# Autodesk Inventor assembly: 0904_right_leg
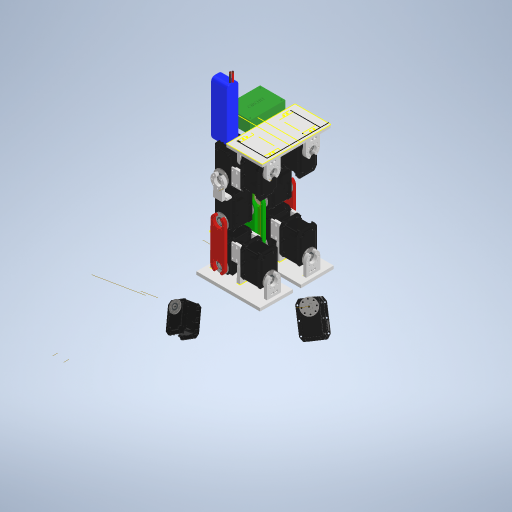
[picture p0: Inventor's stored thumbnail of the model, 512x512]
Saved by Autodesk Inventor 2024.3 (Build 283343000, 343)
## iProperties
Created: 2024-09-03
Part Number: 0904_right_leg
Document SubType Name: Assembly
Designer: gretc
Author: gretc
## Documents named in this file (33)
- C:\Users\gretc\Desktop\inventor_part\0904_right_leg.iam
- C:\Users\gretc\Desktop\inventor_part\다이나믹셀\MX-106T+idle.ipt.iam
- C:\Users\gretc\Desktop\inventor_part\다이나믹셀\MX-64T+idle.ipt.iam
- C:\Users\gretc\Desktop\inventor_part\혼\64-106Horn.ipt
- C:\Users\gretc\Desktop\inventor_part\0904_joint.ipt
- C:\Users\gretc\Desktop\inventor_part\0904_thigh_1.ipt
- C:\Users\gretc\Desktop\inventor_part\0904_thigh_2.ipt
- C:\Users\gretc\Desktop\inventor_part\0904_106-64_adt.ipt
- C:\Users\gretc\Desktop\inventor_part\0904_foot_adt.ipt
- C:\Users\gretc\Desktop\inventor_part\0904_foot-106-adt.ipt
- C:\Users\gretc\Desktop\inventor_part\0904-foot.ipt
- C:\Users\gretc\Desktop\inventor_part\아이들러\64아이들러.iam
- C:\Users\gretc\Desktop\inventor_part\0904-idler-supporter.ipt
- C:\Users\gretc\Desktop\inventor_part\0904_right_foot.ipt
- C:\Users\gretc\Desktop\inventor_part\다이나믹셀\MX-106T+idle.ipt_MIR.iam
- C:\Users\gretc\Desktop\inventor_part\다이나믹셀\MX-64T+idle.ipt_MIR.iam
- C:\Users\gretc\Desktop\inventor_part\혼\64-106Horn_MIR.ipt
- C:\Users\gretc\Desktop\inventor_part\0904_joint_MIR.ipt
- C:\Users\gretc\Desktop\inventor_part\0904_thigh_1_MIR.ipt
- C:\Users\gretc\Desktop\inventor_part\0904_thigh_2_MIR.ipt
- C:\Users\gretc\Desktop\inventor_part\0904_106-64_adt_MIR1.ipt
- C:\Users\gretc\Desktop\inventor_part\0904_foot_adt_MIR.ipt
- C:\Users\gretc\Desktop\inventor_part\아이들러\64아이들러_MIR.iam
- C:\Users\gretc\Desktop\inventor_part\0904-idler-supporter_MIR1.ipt
- C:\Users\gretc\Desktop\inventor_part\0904_right_foot_MIR.ipt
- C:\Users\gretc\Desktop\inventor_part\Power_Control_inventor\Circuit.ipt
- C:\Users\gretc\Desktop\inventor_part\Power_Control_inventor\Enrichpower_2200mAh_11.1V_30C.ipt
- C:\Users\gretc\Desktop\inventor_part\0904_robot_bodyframe1.ipt
- C:\Users\gretc\Desktop\inventor_part\다이나믹셀\MX-28T_R+idle.ipt.iam
- C:\Users\gretc\Desktop\inventor_part\혼\28Horn.ipt
- MX-106T+idle.ipt
- MX-64T+idle.ipt
- MX-28T_R+idle.ipt
## Components (60 placed, 29 different names)
1. MX-106T+idle.ipt:1 [sub-assembly] — 회전:1, 플러쉬:1, 플러쉬:3, 메이트:1, 플러쉬:5, 플러쉬:6, 플러쉬:12, 플러쉬:13, 플러쉬:14, 플러쉬:15, 플러쉬:16
2. MX-64T+idle.ipt:1 [sub-assembly] — 회전:2, 플러쉬:9, 플러쉬:10, 메이트:4, 메이트:15, 삽입:4
3. 64-106Horn:1 — 회전:1, 플러쉬:11, 회전:6
4. 64-106Horn:2 — 회전:2, 삽입:3, 메이트:18, 메이트:21
5. MX-106T+idle.ipt:2 [sub-assembly] — 플러쉬:1, 플러쉬:2, 플러쉬:3, 플러쉬:4, 플러쉬:6, 메이트:2, 플러쉬:9, 플러쉬:10, 메이트:4, 회전:9, 메이트:22, 삽입:5, 메이트:118
6. 64-106Horn:3 — 플러쉬:17
7. MX-106T+idle.ipt:3 [sub-assembly] — 플러쉬:2, 플러쉬:4, 플러쉬:5, 플러쉬:7, 메이트:3, 플러쉬:8, 플러쉬:18, 플러쉬:19, 회전:8, 플러쉬:21, 플러쉬:25, 플러쉬:26, 메이트:25, 메이트:26, 메이트:35
8. 64-106Horn:4 — 메이트:5, 메이트:6, 회전:7
9. 64-106Horn:5 — 회전:5, 메이트:9, 메이트:10, 삽입:1
10. MX-64T+idle.ipt:2 [sub-assembly] — 플러쉬:7, 메이트:3, 플러쉬:8, 회전:5, 플러쉬:20
11. 0904_joint:1 — 플러쉬:11, 플러쉬:12
12. 0904_joint:2 — 회전:6, 회전:7, 각도:2, 플러쉬:29
13. 0904_thigh_1:1 — 플러쉬:13, 플러쉬:14
14. 0904_thigh_2:1 — 플러쉬:15, 플러쉬:16, 플러쉬:17
15. 0904_106-64_adt:1 — 플러쉬:18, 플러쉬:19
16. 0904_foot_adt:1 — 플러쉬:20, 플러쉬:23, 플러쉬:24
17. 0904_106-64_adt:2 — 회전:8
18. 0904_106-64_adt:3 — 회전:9
19. 0904_foot_adt:2 — 삽입:1, 플러쉬:27, 플러쉬:28
20. 0904_foot-106-adt:1 — 플러쉬:21
21. 0904_foot_adt:4 — 삽입:3, 메이트:19, 플러쉬:22
22. 0904_foot_adt:5 — 삽입:4, 메이트:16, 플러쉬:22
23. 0904_106-64_adt:4 — 메이트:23, 삽입:5
24. 0904-foot:1 — 플러쉬:23, 플러쉬:24
25. 64아이들러:1 [sub-assembly] — 메이트:28, 메이트:29, 메이트:30, 메이트:31, 메이트:32, 메이트:38, 삽입:6, 메이트:43, 메이트:45
26. 0904-idler-supporter:1 — 플러쉬:25, 플러쉬:26, 메이트:27, 메이트:29
27. 0904_foot_adt:6 — 메이트:40, 삽입:6, 각도:2, 메이트:48
28. 0904_right_foot:1 — 플러쉬:27, 플러쉬:28
29. MX-106T+idle.ipt_MIR:1 [sub-assembly] — 메이트:72, 플러쉬:33, 플러쉬:34, 플러쉬:35, 플러쉬:36, 메이트:77, 메이트:79, 메이트:80, 메이트:82, 메이트:83, 회전:10
30. MX-64T+idle.ipt_MIR:1 [sub-assembly] — 메이트:73, 플러쉬:30, 플러쉬:31, 메이트:87, 삽입:8, 회전:11
31. 64-106Horn_MIR:1 — 메이트:78, 회전:10, 회전:15
32. 64-106Horn_MIR:2 — 삽입:7, 메이트:90, 메이트:93, 회전:11
33. MX-106T+idle.ipt_MIR:2 [sub-assembly] — 메이트:73, 플러쉬:30, 플러쉬:31, 플러쉬:32, 플러쉬:33, 플러쉬:34, 플러쉬:35, 플러쉬:37, 플러쉬:38, 삽입:9, 메이트:94, 회전:12, 회전:17, 메이트:119
34. 64-106Horn_MIR:3 — 메이트:81, 회전:12
35. MX-106T+idle.ipt_MIR:3 [sub-assembly] — 플러쉬:36, 플러쉬:37, 플러쉬:38, 플러쉬:39, 메이트:74, 플러쉬:40, 메이트:84, 메이트:85, 메이트:98, 메이트:99, 메이트:100, 메이트:101, 메이트:107, 회전:13, 회전:16
36. 64-106Horn_MIR:4 — 메이트:75, 메이트:76, 회전:13, 회전:14
37. MX-64T+idle.ipt_MIR:2 [sub-assembly] — 플러쉬:39, 메이트:74, 플러쉬:40, 메이트:86
38. 0904_joint_MIR:1 — 메이트:77, 메이트:78
39. 0904_joint_MIR:2 — 각도:3, 메이트:117, 회전:14, 회전:15
40. 0904_thigh_1_MIR:1 — 메이트:79, 메이트:80
41. 0904_thigh_2_MIR:1 — 메이트:81, 메이트:82, 메이트:83
42. 0904_106-64_adt_MIR1:1 — 메이트:84, 메이트:85
43. 0904_foot_adt_MIR:1 — 메이트:86
44. 0904_106-64_adt_MIR1:2 — 회전:16
45. 0904_106-64_adt_MIR1:3 — 회전:17
46. 0904_foot_adt_MIR:2 — 메이트:115, 메이트:116
47. 0904_foot_adt_MIR:3 — 삽입:7, 플러쉬:41, 메이트:92, 플러쉬:42, 플러쉬:43
48. 0904_foot_adt_MIR:4 — 플러쉬:41, 삽입:8, 메이트:89
49. 0904_106-64_adt_MIR1:4 — 삽입:9, 메이트:96
50. 64아이들러_MIR:1 [sub-assembly] — 메이트:97, 메이트:103, 메이트:104, 메이트:105, 메이트:106, 삽입:10, 메이트:108, 메이트:111, 메이트:113
51. 0904-idler-supporter_MIR1:1 — 메이트:97, 메이트:98, 메이트:99, 메이트:102
52. 0904_foot_adt_MIR:5 — 각도:3, 삽입:10, 메이트:109, 메이트:114
53. 0904_right_foot_MIR:1 — 메이트:115, 메이트:116
54. Circuit:1 — 메이트:118
55. Enrichpower_2200mAh_11.1V_30C:1 — 메이트:119
56. 0904_robot_bodyframe1:1 — 플러쉬:42, 플러쉬:43
57. MX-28T_R+idle.ipt:1 [sub-assembly] — 메이트:120, 메이트:123
58. MX-64T+idle.ipt:3 [sub-assembly] — 메이트:129, 메이트:132
59. 28Horn:1 — 메이트:121, 메이트:123, 메이트:124
60. 64-106Horn:6 — 메이트:130, 메이트:132
## Relationships (165: Mate 92, Flush 43, RevoluteJoint 17, Insert 9, Angle 4)
- 회전:1 [RevoluteJoint]: MX-106T+idle.ipt:1 ↔ 64-106Horn:1
- 회전:2 [RevoluteJoint]: MX-64T+idle.ipt:1 ↔ 64-106Horn:2
- [RevoluteJoint]: MX-106T+idle.ipt:2 ↔ 64-106Horn:3
- [RevoluteJoint]: MX-106T+idle.ipt:3 ↔ 64-106Horn:4
- 플러쉬:1 [Flush]: MX-106T+idle.ipt:1 ↔ MX-106T+idle.ipt:2
- 플러쉬:2 [Flush]: MX-106T+idle.ipt:2 ↔ MX-106T+idle.ipt:3
- 플러쉬:3 [Flush]: MX-106T+idle.ipt:1 ↔ MX-106T+idle.ipt:2
- 플러쉬:4 [Flush]: MX-106T+idle.ipt:2 ↔ MX-106T+idle.ipt:3
- 메이트:1 [Mate]: MX-106T+idle.ipt:1
- 플러쉬:5 [Flush] (75 mm): MX-106T+idle.ipt:1 ↔ MX-106T+idle.ipt:3
- 플러쉬:6 [Flush] (75 mm): MX-106T+idle.ipt:1 ↔ MX-106T+idle.ipt:2
- 메이트:2 [Mate]: MX-106T+idle.ipt:2
- 플러쉬:7 [Flush]: MX-106T+idle.ipt:3 ↔ MX-64T+idle.ipt:2
- 메이트:3 [Mate]: MX-106T+idle.ipt:3 ↔ MX-64T+idle.ipt:2
- 플러쉬:8 [Flush] (50 mm): MX-106T+idle.ipt:3 ↔ MX-64T+idle.ipt:2
- 회전:5 [RevoluteJoint]: 64-106Horn:5 ↔ MX-64T+idle.ipt:2
- 플러쉬:9 [Flush]: MX-64T+idle.ipt:1 ↔ MX-106T+idle.ipt:2
- 플러쉬:10 [Flush] (50 mm): MX-64T+idle.ipt:1 ↔ MX-106T+idle.ipt:2
- 메이트:4 [Mate] (-35 mm): MX-64T+idle.ipt:1 ↔ MX-106T+idle.ipt:2
- 메이트:5 [Mate]: 64-106Horn:4
- 메이트:6 [Mate]: 64-106Horn:4
- 플러쉬:11 [Flush]: 64-106Horn:1 ↔ 0904_joint:1
- 플러쉬:12 [Flush]: MX-106T+idle.ipt:1 ↔ 0904_joint:1
- 회전:6 [RevoluteJoint]: 64-106Horn:1 ↔ 0904_joint:2
- 회전:7 [RevoluteJoint]: 64-106Horn:4 ↔ 0904_joint:2
- 플러쉬:13 [Flush]: MX-106T+idle.ipt:1 ↔ 0904_thigh_1:1
- 플러쉬:14 [Flush]: MX-106T+idle.ipt:1 ↔ 0904_thigh_1:1
- 플러쉬:15 [Flush]: MX-106T+idle.ipt:1 ↔ 0904_thigh_2:1
- 플러쉬:16 [Flush]: MX-106T+idle.ipt:1 ↔ 0904_thigh_2:1
- 플러쉬:17 [Flush]: 64-106Horn:3 ↔ 0904_thigh_2:1
- 플러쉬:18 [Flush]: MX-106T+idle.ipt:3 ↔ 0904_106-64_adt:1
- 플러쉬:19 [Flush]: MX-106T+idle.ipt:3 ↔ 0904_106-64_adt:1
- 플러쉬:20 [Flush]: MX-64T+idle.ipt:2 ↔ 0904_foot_adt:1
- 회전:8 [RevoluteJoint]: MX-106T+idle.ipt:3 ↔ 0904_106-64_adt:2
- 회전:9 [RevoluteJoint]: MX-106T+idle.ipt:2 ↔ 0904_106-64_adt:3
- 메이트:9 [Mate]: 64-106Horn:5
- 메이트:10 [Mate]: 64-106Horn:5
- 삽입:1 [Insert] (-1.5 mm): 64-106Horn:5 ↔ 0904_foot_adt:2
- 플러쉬:21 [Flush]: MX-106T+idle.ipt:3 ↔ 0904_foot-106-adt:1
- 삽입:3 [Insert] (-1.5 mm): 64-106Horn:2 ↔ 0904_foot_adt:4
- 메이트:15 [Mate]: MX-64T+idle.ipt:1
- 삽입:4 [Insert]: MX-64T+idle.ipt:1 ↔ 0904_foot_adt:5
- 메이트:16 [Mate]: 0904_foot_adt:5
- 메이트:17 [Mate]
- 메이트:18 [Mate]: 64-106Horn:2
- 메이트:19 [Mate]: 0904_foot_adt:4
- 메이트:20 [Mate]
- 메이트:21 [Mate]: 64-106Horn:2
- 플러쉬:22 [Flush]: 0904_foot_adt:4 ↔ 0904_foot_adt:5
- 메이트:22 [Mate]: MX-106T+idle.ipt:2
- 메이트:23 [Mate]: 0904_106-64_adt:4
- 메이트:24 [Mate]
- 삽입:5 [Insert]: MX-106T+idle.ipt:2 ↔ 0904_106-64_adt:4
- 플러쉬:23 [Flush]: 0904_foot_adt:1 ↔ 0904-foot:1
- 플러쉬:24 [Flush]: 0904_foot_adt:1 ↔ 0904-foot:1
- 플러쉬:25 [Flush]: MX-106T+idle.ipt:3 ↔ 0904-idler-supporter:1
- 플러쉬:26 [Flush]: MX-106T+idle.ipt:3 ↔ 0904-idler-supporter:1
- 메이트:25 [Mate]: MX-106T+idle.ipt:3
- 메이트:26 [Mate]: MX-106T+idle.ipt:3
- 메이트:27 [Mate]: 0904-idler-supporter:1
- 메이트:28 [Mate]: 64아이들러:1
- 메이트:29 [Mate]: 64아이들러:1 ↔ 0904-idler-supporter:1
- 메이트:30 [Mate]: 64아이들러:1
- 메이트:31 [Mate]: 64아이들러:1
- 메이트:32 [Mate]: 64아이들러:1
- 메이트:35 [Mate]: MX-106T+idle.ipt:3
- 각도:1 [Angle] (0 deg)
- 메이트:38 [Mate]: 64아이들러:1
- 메이트:40 [Mate]: 0904_foot_adt:6
- 삽입:6 [Insert] (0.76 mm): 64아이들러:1 ↔ 0904_foot_adt:6
- 메이트:43 [Mate]: 64아이들러:1
- 메이트:44 [Mate]
- 메이트:45 [Mate]: 64아이들러:1
- 메이트:46 [Mate]
- 각도:2 [Angle] (0 deg): 0904_joint:2 ↔ 0904_foot_adt:6
- 메이트:48 [Mate]: 0904_foot_adt:6
- 플러쉬:27 [Flush]: 0904_foot_adt:2 ↔ 0904_right_foot:1
- 플러쉬:28 [Flush]: 0904_foot_adt:2 ↔ 0904_right_foot:1
- 메이트:71 [Mate]
- 플러쉬:29 [Flush] (5 mm): 0904_joint:2
- 메이트:72 [Mate]: MX-106T+idle.ipt_MIR:1
- 메이트:73 [Mate] (35 mm): MX-64T+idle.ipt_MIR:1 ↔ MX-106T+idle.ipt_MIR:2
- 플러쉬:30 [Flush] (-50 mm): MX-64T+idle.ipt_MIR:1 ↔ MX-106T+idle.ipt_MIR:2
- 플러쉬:31 [Flush]: MX-64T+idle.ipt_MIR:1 ↔ MX-106T+idle.ipt_MIR:2
- 플러쉬:32 [Flush]: MX-106T+idle.ipt_MIR:2
- 플러쉬:33 [Flush] (-75 mm): MX-106T+idle.ipt_MIR:1 ↔ MX-106T+idle.ipt_MIR:2
- 플러쉬:34 [Flush]: MX-106T+idle.ipt_MIR:1 ↔ MX-106T+idle.ipt_MIR:2
- 플러쉬:35 [Flush]: MX-106T+idle.ipt_MIR:1 ↔ MX-106T+idle.ipt_MIR:2
- 플러쉬:36 [Flush] (-75 mm): MX-106T+idle.ipt_MIR:1 ↔ MX-106T+idle.ipt_MIR:3
- 플러쉬:37 [Flush]: MX-106T+idle.ipt_MIR:2 ↔ MX-106T+idle.ipt_MIR:3
- 플러쉬:38 [Flush]: MX-106T+idle.ipt_MIR:2 ↔ MX-106T+idle.ipt_MIR:3
- 플러쉬:39 [Flush] (-50 mm): MX-106T+idle.ipt_MIR:3 ↔ MX-64T+idle.ipt_MIR:2
- 메이트:74 [Mate]: MX-106T+idle.ipt_MIR:3 ↔ MX-64T+idle.ipt_MIR:2
- 플러쉬:40 [Flush]: MX-106T+idle.ipt_MIR:3 ↔ MX-64T+idle.ipt_MIR:2
- 메이트:75 [Mate]: 64-106Horn_MIR:4
- 메이트:76 [Mate]: 64-106Horn_MIR:4
- 메이트:77 [Mate]: MX-106T+idle.ipt_MIR:1 ↔ 0904_joint_MIR:1
- 메이트:78 [Mate]: 64-106Horn_MIR:1 ↔ 0904_joint_MIR:1
- 메이트:79 [Mate]: MX-106T+idle.ipt_MIR:1 ↔ 0904_thigh_1_MIR:1
- 메이트:80 [Mate]: MX-106T+idle.ipt_MIR:1 ↔ 0904_thigh_1_MIR:1
- 메이트:81 [Mate]: 64-106Horn_MIR:3 ↔ 0904_thigh_2_MIR:1
- 메이트:82 [Mate]: MX-106T+idle.ipt_MIR:1 ↔ 0904_thigh_2_MIR:1
- 메이트:83 [Mate]: MX-106T+idle.ipt_MIR:1 ↔ 0904_thigh_2_MIR:1
- 메이트:84 [Mate]: MX-106T+idle.ipt_MIR:3 ↔ 0904_106-64_adt_MIR1:1
- 메이트:85 [Mate]: MX-106T+idle.ipt_MIR:3 ↔ 0904_106-64_adt_MIR1:1
- 메이트:86 [Mate]: MX-64T+idle.ipt_MIR:2 ↔ 0904_foot_adt_MIR:1
- 삽입:7 [Insert] (-1.5 mm): 64-106Horn_MIR:2 ↔ 0904_foot_adt_MIR:3
- 메이트:87 [Mate]: MX-64T+idle.ipt_MIR:1
- 플러쉬:41 [Flush]: 0904_foot_adt_MIR:3 ↔ 0904_foot_adt_MIR:4
- 삽입:8 [Insert]: MX-64T+idle.ipt_MIR:1 ↔ 0904_foot_adt_MIR:4
- 메이트:88 [Mate]
- 메이트:89 [Mate]: 0904_foot_adt_MIR:4
- 메이트:90 [Mate]: 64-106Horn_MIR:2
- 메이트:91 [Mate]
- 메이트:92 [Mate]: 0904_foot_adt_MIR:3
- 메이트:93 [Mate]: 64-106Horn_MIR:2
- 삽입:9 [Insert]: MX-106T+idle.ipt_MIR:2 ↔ 0904_106-64_adt_MIR1:4
- 메이트:94 [Mate]: MX-106T+idle.ipt_MIR:2
- 메이트:95 [Mate]
- 메이트:96 [Mate]: 0904_106-64_adt_MIR1:4
- 메이트:97 [Mate]: 64아이들러_MIR:1 ↔ 0904-idler-supporter_MIR1:1
- 메이트:98 [Mate]: MX-106T+idle.ipt_MIR:3 ↔ 0904-idler-supporter_MIR1:1
- 메이트:99 [Mate]: MX-106T+idle.ipt_MIR:3 ↔ 0904-idler-supporter_MIR1:1
- 메이트:100 [Mate]: MX-106T+idle.ipt_MIR:3
- 메이트:101 [Mate]: MX-106T+idle.ipt_MIR:3
- 메이트:102 [Mate]: 0904-idler-supporter_MIR1:1
- 메이트:103 [Mate]: 64아이들러_MIR:1
- 메이트:104 [Mate]: 64아이들러_MIR:1
- 메이트:105 [Mate]: 64아이들러_MIR:1
- 메이트:106 [Mate]: 64아이들러_MIR:1
- 각도:3 [Angle] (0 deg): 0904_joint_MIR:2 ↔ 0904_foot_adt_MIR:5
- 삽입:10 [Insert] (0.76 mm): 64아이들러_MIR:1 ↔ 0904_foot_adt_MIR:5
- 메이트:107 [Mate]: MX-106T+idle.ipt_MIR:3
- 각도:4 [Angle] (0 deg)
- 메이트:108 [Mate]: 64아이들러_MIR:1
- 메이트:109 [Mate]: 0904_foot_adt_MIR:5
- 메이트:110 [Mate]
- 메이트:111 [Mate]: 64아이들러_MIR:1
- 메이트:112 [Mate]
- 메이트:113 [Mate]: 64아이들러_MIR:1
- 메이트:114 [Mate]: 0904_foot_adt_MIR:5
- 메이트:115 [Mate]: 0904_foot_adt_MIR:2 ↔ 0904_right_foot_MIR:1
- 메이트:116 [Mate]: 0904_foot_adt_MIR:2 ↔ 0904_right_foot_MIR:1
- 메이트:117 [Mate] (5 mm): 0904_joint_MIR:2
- 회전:10 [RevoluteJoint]: MX-106T+idle.ipt_MIR:1 ↔ 64-106Horn_MIR:1
- 회전:11 [RevoluteJoint]: MX-64T+idle.ipt_MIR:1 ↔ 64-106Horn_MIR:2
- 회전:12 [RevoluteJoint]: MX-106T+idle.ipt_MIR:2 ↔ 64-106Horn_MIR:3
- 회전:13 [RevoluteJoint]: MX-106T+idle.ipt_MIR:3 ↔ 64-106Horn_MIR:4
- 회전:14 [RevoluteJoint]: 64-106Horn_MIR:4 ↔ 0904_joint_MIR:2
- 회전:15 [RevoluteJoint]: 64-106Horn_MIR:1 ↔ 0904_joint_MIR:2
- 회전:16 [RevoluteJoint]: MX-106T+idle.ipt_MIR:3 ↔ 0904_106-64_adt_MIR1:2
- 회전:17 [RevoluteJoint]: MX-106T+idle.ipt_MIR:2 ↔ 0904_106-64_adt_MIR1:3
- 플러쉬:42 [Flush]: 0904_foot_adt_MIR:3 ↔ 0904_robot_bodyframe1:1
- 플러쉬:43 [Flush]: 0904_foot_adt_MIR:3 ↔ 0904_robot_bodyframe1:1
- 메이트:118 [Mate]: MX-106T+idle.ipt:2 ↔ Circuit:1
- 메이트:119 [Mate]: MX-106T+idle.ipt_MIR:2 ↔ Enrichpower_2200mAh_11.1V_30C:1
- 메이트:120 [Mate]: MX-28T_R+idle.ipt:1
- 메이트:121 [Mate]: 28Horn:1
- 메이트:122 [Mate]
- 메이트:123 [Mate]: MX-28T_R+idle.ipt:1 ↔ 28Horn:1
- 메이트:124 [Mate]: 28Horn:1
- 메이트:129 [Mate]: MX-64T+idle.ipt:3
- 메이트:130 [Mate]: 64-106Horn:6
- 메이트:131 [Mate]
- 메이트:132 [Mate]: MX-64T+idle.ipt:3 ↔ 64-106Horn:6
## Named parameters: d14_d10 = 0 mm, d15_d11 = -179.999728 deg, d16_d10 = 0 mm, d17_d11 = -135 deg
